# Autodesk Inventor assembly: Idler Assembly
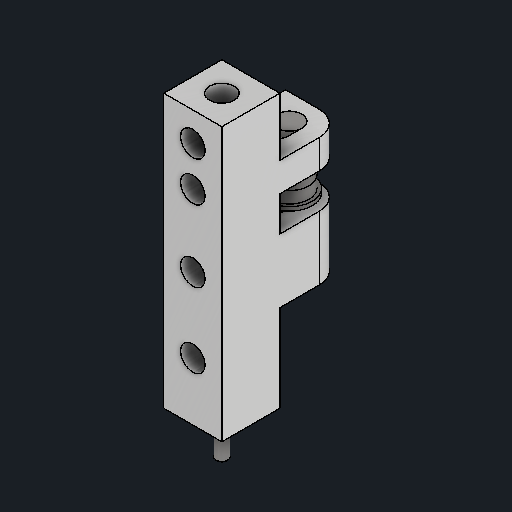
[picture p0: Inventor's stored thumbnail of the model, 512x512]
Saved by Autodesk Inventor 2026.2 (Build 302298000, 298)
## iProperties
Created: 2025-05-27
Part Number: Idler Assembly
Document SubType Name: Assembly
Designer: Joshua Eah
Author: Joshua Eah
## Documents named in this file (7)
- C:\Users\JoshuaEah\Documents\GitHub\Voron-0\CAD\Idlers\B Idler Assembly.iam
- C:\Users\JoshuaEah\Documents\GitHub\Voron-0\CAD\Hardware\Bearings\F623 Stack.iam
- C:\Users\JoshuaEah\Documents\GitHub\Voron-0\CAD\Idlers\Bearing Nut.ipt
- C:\Users\JoshuaEah\Documents\GitHub\Voron-0\CAD\Hardware\Pins\3x12 Pin.ipt
- C:\Users\JoshuaEah\Documents\GitHub\Voron-0\CAD\Hardware\Fasteners\M3x20 SHCS.ipt
- C:\Users\JoshuaEah\Documents\GitHub\Voron-0\CAD\Hardware\Fasteners\M3x10 BHCS.ipt
- C:\Users\JoshuaEah\Documents\GitHub\Voron-0\CAD\Idlers\B Idler.ipt
## Components (10 placed, 6 different names)
1. B Idler:1 — Insert:3, Insert:4, Insert:5, Insert:6, Insert:7, Mate:11
2. Bearing Nut:1 — Mate:6, Insert:2, Mate:10
3. Bearing Nut:2 — Mate:5, Insert:1, Mate:9, Mate:11
4. 3x12 Pin:1 — Mate:5, Mate:6, Insert:1
5. F623 Stack:1 [sub-assembly] — Insert:2
6. M3x20 SHCS:1 — Insert:3, Mate:9
7. M3x20 SHCS:3 — Insert:6, Mate:10
8. M3x10 BHCS:1 — Insert:4
9. M3x10 BHCS:2 — Insert:7
10. M3x20 SHCS:2 — Insert:5
## Relationships (12: Insert 7, Mate 5)
- Mate:5: Bearing Nut:2 ↔ 3x12 Pin:1
- Mate:6: Bearing Nut:1 ↔ 3x12 Pin:1
- Insert:1: Bearing Nut:2 ↔ 3x12 Pin:1
- Insert:2: Bearing Nut:1 ↔ F623 Stack:1
- Insert:3: B Idler:1 ↔ M3x20 SHCS:1
- Insert:4: B Idler:1 ↔ M3x10 BHCS:1
- Insert:5: B Idler:1 ↔ M3x20 SHCS:2
- Mate:9: Bearing Nut:2 ↔ M3x20 SHCS:1
- Insert:6: B Idler:1 ↔ M3x20 SHCS:3
- Mate:10: Bearing Nut:1 ↔ M3x20 SHCS:3
- Insert:7: B Idler:1 ↔ M3x10 BHCS:2
- Mate:11: B Idler:1 ↔ Bearing Nut:2
